# Autodesk Inventor assembly: test-model-2025a
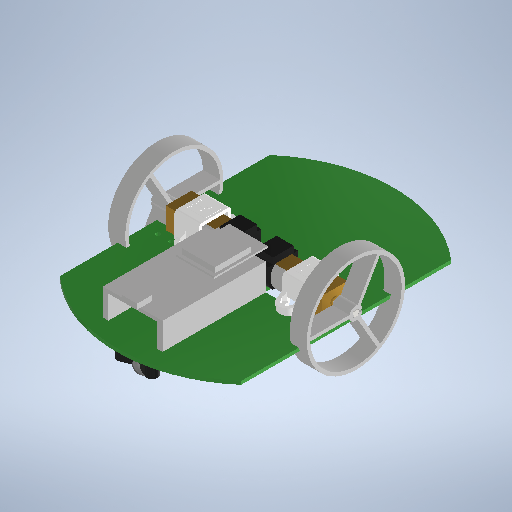
[picture p0: Inventor's stored thumbnail of the model, 512x512]
Saved by Autodesk Inventor 2025.3 (Build 293356000, 356)
## iProperties
Created: 2025-05-26
Part Number: test-model-2025a
Document SubType Name: Assembly
Designer: yamashita1
Author: yamashita1
## Documents named in this file (7)
- G:\マイドライブ\project\micro-mouse\3D-Model\test-model-2025a.iam
- G:\マイドライブ\project\micro-mouse\3D-Model\BaseBoard1.ipt
- G:\マイドライブ\project\micro-mouse\3D-Model\N20withBracket.iam
- G:\マイドライブ\project\micro-mouse\3D-Model\BallCaster-H16.ipt
- G:\マイドライブ\project\micro-mouse\3D-Model\Ground.ipt
- G:\マイドライブ\project\micro-mouse\3D-Model\D-Shaft_Wheel2.ipt
- G:\マイドライブ\project\micro-mouse\3D-Model\ESP32-DevKitC.ipt
## Components (9 placed, 6 different names)
1. BaseBoard1:1 — メイト:1, メイト:2, メイト:3, メイト:4, メイト:5
2. N20withBracket:1 [sub-assembly] — メイト:2, メイト:6, メイト:7
3. N20withBracket:2 [sub-assembly] — メイト:1, メイト:8
4. BallCaster-H16:1 — メイト:3
5. BallCaster-H16:2 — メイト:4
6. Ground:1 — メイト:5
7. D-Shaft_Wheel2:1 — メイト:8
8. D-Shaft_Wheel2:2 — メイト:6, メイト:7
9. ESP32-DevKitC:1
## Relationships (8: Mate 8)
- メイト:1 [Mate]: BaseBoard1:1 ↔ N20withBracket:2
- メイト:2 [Mate]: BaseBoard1:1 ↔ N20withBracket:1
- メイト:3 [Mate]: BaseBoard1:1 ↔ BallCaster-H16:1
- メイト:4 [Mate]: BaseBoard1:1 ↔ BallCaster-H16:2
- メイト:5 [Mate] (16 mm): BaseBoard1:1 ↔ Ground:1
- メイト:6 [Mate]: N20withBracket:1 ↔ D-Shaft_Wheel2:2
- メイト:7 [Mate]: N20withBracket:1 ↔ D-Shaft_Wheel2:2
- メイト:8 [Mate]: N20withBracket:2 ↔ D-Shaft_Wheel2:1
